# Autodesk Inventor assembly: patio
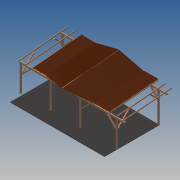
[picture p0: Inventor's stored thumbnail of the model, 180x180]
Saved by Autodesk Inventor 2013 (Build 170138000, 138)
## iProperties
Created: 2013-08-10
Part Number: patio
Document SubType Name: Assembly
Designer: ddeboer
Author: ddeboer
## Documents named in this file (10)
- C:\Users\ddeboer\Desktop\patio\patio.iam
- C:\Users\ddeboer\Desktop\patio\slab.ipt
- C:\Users\ddeboer\Desktop\patio\highSide.ipt
- C:\Users\ddeboer\Desktop\patio\lowSide.ipt
- C:\Users\ddeboer\Desktop\patio\peak.ipt
- C:\Users\ddeboer\Desktop\patio\beam.ipt
- C:\Users\ddeboer\Desktop\patio\roofPanel1.iam
- C:\Users\ddeboer\Desktop\patio\roofPanel2.iam
- C:\Users\ddeboer\Desktop\patio\roofPanel3.iam
- C:\Users\ddeboer\Desktop\patio\gableSupport.ipt
## Components (11 placed, 9 different names)
1. slab:1 — Insert:1, Insert:2
2. highSide:1 — Insert:1, Mate:2
3. lowSide:1 — Insert:2, Mate:1
4. peak:1 — Mate:1, Mate:4
5. peak:2 — Mate:2, Mate:3
6. beam:1 — Mate:3
7. roofPanel1:1 [sub-assembly]
8. roofPanel1:2 [sub-assembly]
9. roofPanel2:1 [sub-assembly]
10. roofPanel3:1 [sub-assembly]
11. gableSupport:1 — Mate:4
## Relationships (6: Mate 4, Insert 2)
- Insert:1: slab:1 ↔ highSide:1
- Insert:2: slab:1 ↔ lowSide:1
- Mate:1: lowSide:1 ↔ peak:1
- Mate:2: highSide:1 ↔ peak:2
- Mate:3: peak:2 ↔ beam:1
- Mate:4: peak:1 ↔ gableSupport:1
